# Autodesk Inventor assembly: PIP_Main Unit Subassembly
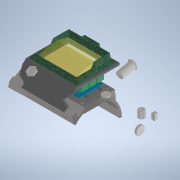
[picture p0: Inventor's stored thumbnail of the model, 180x180]
Saved by Autodesk Inventor 2021 (Build 250183000, 183)
## iProperties
Created: 2021-05-26
Part Number: PIP_Main Unit Subassembly
Document SubType Name: Assembly
Designer: trent
Author: trent
## Documents named in this file (11)
- C:\Users\EmeraldLeeTiger\OneDrive - wmpenn.edu\Personal\PIP-Boy 6400 Mk.I\PIP_Main Unit Subassembly.iam
- C:\Users\EmeraldLeeTiger\OneDrive - wmpenn.edu\Personal\PIP-Boy 6400 Mk.I\MainHousing_FrontMainShell.ipt
- C:\Users\EmeraldLeeTiger\OneDrive - wmpenn.edu\Personal\PIP-Boy 6400 Mk.I\MainHousing_Screen Acrylic.ipt
- C:\Users\EmeraldLeeTiger\OneDrive - wmpenn.edu\Personal\PIP-Boy 6400 Mk.I\MainHousing_Screen Visor.ipt
- C:\Users\EmeraldLeeTiger\OneDrive - wmpenn.edu\Personal\PIP-Boy 6400 Mk.I\MainHousing_BackMainShell.ipt
- C:\Users\EmeraldLeeTiger\OneDrive - wmpenn.edu\Personal\PIP-Boy 6400 Mk.I\PIP-Boy 6400 Mk_I Computer Subassembly.iam
- C:\Users\EmeraldLeeTiger\OneDrive - wmpenn.edu\Personal\PIP-Boy 6400 Mk.I\16mmToggleButton.ipt
- C:\Users\EmeraldLeeTiger\OneDrive - wmpenn.edu\Personal\PIP-Boy 6400 Mk.I\Button_SelectButton.ipt
- C:\Users\EmeraldLeeTiger\OneDrive - wmpenn.edu\Personal\PIP-Boy 6400 Mk.I\Dial_InventoryScroll.ipt
- C:\Users\EmeraldLeeTiger\OneDrive - wmpenn.edu\Personal\PIP-Boy 6400 Mk.I\Dial_Radio.ipt
- C:\Users\EmeraldLeeTiger\OneDrive - wmpenn.edu\Personal\PIP-Boy 6400 Mk.I\Dial_Main-Sub Menu Dial.ipt
## Components (11 placed, 10 different names)
1. MainHousing_FrontMainShell:1 — Mate:1, Mate:2, Mate:3, Mate:4, Mate:5, Mate:6, Mate:10, Mate:11, Mate:13, Mate:14
2. MainHousing_Screen Acrylic:1 — Mate:1, Mate:2, Mate:3, Mate:12
3. MainHousing_Screen Visor:1 — Mate:4, Mate:5, Mate:6
4. MainHousing_BackMainShell:1 — Mate:7, Mate:8, Mate:9
5. PIP-Boy 6400 Mk_I Computer Subassembly:1 [sub-assembly] — Mate:7, Mate:8, Mate:9, Mate:10, Mate:11, Mate:12
6. 16mmToggleButton:1
7. 16mmToggleButton:2 — Mate:13, Mate:14
8. Button_SelectButton:1
9. Dial_InventoryScroll:1
10. Dial_Radio:1
11. Dial_Main-Sub Menu Dial:1
## Relationships (14: Mate 14)
- Mate:1: MainHousing_FrontMainShell:1 ↔ MainHousing_Screen Acrylic:1
- Mate:2: MainHousing_FrontMainShell:1 ↔ MainHousing_Screen Acrylic:1
- Mate:3: MainHousing_FrontMainShell:1 ↔ MainHousing_Screen Acrylic:1
- Mate:4: MainHousing_FrontMainShell:1 ↔ MainHousing_Screen Visor:1
- Mate:5: MainHousing_FrontMainShell:1 ↔ MainHousing_Screen Visor:1
- Mate:6: MainHousing_FrontMainShell:1 ↔ MainHousing_Screen Visor:1
- Mate:7: MainHousing_BackMainShell:1 ↔ PIP-Boy 6400 Mk_I Computer Subassembly:1
- Mate:8: MainHousing_BackMainShell:1 ↔ PIP-Boy 6400 Mk_I Computer Subassembly:1
- Mate:9: MainHousing_BackMainShell:1 ↔ PIP-Boy 6400 Mk_I Computer Subassembly:1
- Mate:10 (1 mm): MainHousing_FrontMainShell:1 ↔ PIP-Boy 6400 Mk_I Computer Subassembly:1
- Mate:11 (7 mm): MainHousing_FrontMainShell:1 ↔ PIP-Boy 6400 Mk_I Computer Subassembly:1
- Mate:12 (2.5 mm): MainHousing_Screen Acrylic:1 ↔ PIP-Boy 6400 Mk_I Computer Subassembly:1
- Mate:13: MainHousing_FrontMainShell:1 ↔ 16mmToggleButton:2
- Mate:14: MainHousing_FrontMainShell:1 ↔ 16mmToggleButton:2
